# Autodesk Inventor assembly: robot
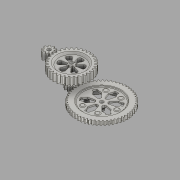
[picture p0: Inventor's stored thumbnail of the model, 180x180]
Saved by Autodesk Inventor 2020 (Build 240168000, 168)
## iProperties
Created: 2020-07-14
Part Number: robot
Document SubType Name: Assembly
Designer: alons
Author: alons
## Documents named in this file (5)
- C:\Users\alons\OneDrive\Documents\GitHub\Water-Strider-Robot\Striderbot\robot.iam
- C:\Users\alons\OneDrive\Documents\GitHub\Water-Strider-Robot\Striderbot\spur_gears_mesh_2\Design Accelerator\Spur Gear13.ipt
- C:\Users\alons\OneDrive\Documents\GitHub\Water-Strider-Robot\Striderbot\spur_gears_mesh_2\Design Accelerator\Spur Gear23.ipt
- C:\Users\alons\OneDrive\Documents\GitHub\Water-Strider-Robot\Striderbot\spur_gears_mesh_3\Design Accelerator\Spur Gear11.ipt
- C:\Users\alons\OneDrive\Documents\GitHub\Water-Strider-Robot\Striderbot\spur_gears_mesh_3\Design Accelerator\Spur Gear21.ipt
## Components (4 placed, 2 different names)
1. Spur Gear1:1 — Mate:1, Mate:2, Flush:1, Mate:3, Rotation:1
2. Spur Gear2:1 — Flush:1, Mate:3, Mate:4, Rotation:1, Flush:2, Mate:6
3. Spur Gear1:2 — Mate:5, Flush:2, Mate:6, Flush:3, Mate:7, Rotation:3
4. Spur Gear2:2 — Flush:3, Mate:7, Mate:8, Rotation:3
## Relationships (13: Mate 8, Flush 3, RelateRotation 2)
- Mate:1 (-20 mm): Spur Gear1:1
- Mate:2: Spur Gear1:1
- Flush:1: Spur Gear1:1 ↔ Spur Gear2:1
- Mate:3 (6.3 mm): Spur Gear1:1 ↔ Spur Gear2:1
- Mate:4: Spur Gear2:1
- Rotation:1 [RelateRotation] (0.2812 ul): Spur Gear1:1 ↔ Spur Gear2:1
- Mate:5 (-25 mm): Spur Gear1:2
- Flush:2: Spur Gear2:1 ↔ Spur Gear1:2
- Mate:6: Spur Gear2:1 ↔ Spur Gear1:2
- Flush:3: Spur Gear1:2 ↔ Spur Gear2:2
- Mate:7 (8.45 mm): Spur Gear1:2 ↔ Spur Gear2:2
- Mate:8: Spur Gear2:2
- Rotation:3 [RelateRotation] (5.689 ul): Spur Gear1:2 ↔ Spur Gear2:2
